# Autodesk Inventor assembly: ExtruderQuickReleaseRight
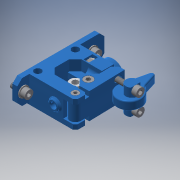
[picture p0: Inventor's stored thumbnail of the model, 180x180]
Saved by Autodesk Inventor 2016 (Build 200138000, 138)
## iProperties
Created: 2015-05-07
Part Number: ExtruderQuickReleaseRight
Document SubType Name: Assembly
Designer: Jack
Author: Jack
## Documents named in this file (14)
- C:\Users\Jack\ownCloud\Projects\CrossBot\InventorModel\Extruder\ExtruderQuickRelease\ExtruderQuickReleaseRight.iam
- C:\Users\Jack\ownCloud\Projects\CrossBot\InventorModel\Extruder\ExtruderQuickRelease\ExtruderQuickReleaseBodyRight.ipt
- C:\Users\Jack\ownCloud\Projects\CrossBot\InventorModel\Extruder\ExtruderQuickRelease\ExtruderQuickReleaseIdlerRight.ipt
- C:\Users\Jack\ownCloud\Projects\CrossBot\InventorModel\Extruder\ExtruderQuickRelease\ExtruderQuickReleaseTensionCam.ipt
- C:\Users\Jack\ownCloud\Projects\CrossBot\InventorModel\Extruder\ExtruderQuickRelease\ExtruderQuickReleaseTensionDowel.ipt
- C:\Users\Jack\ownCloud\Projects\CrossBot\InventorModel\Electronics\Motors\StepperMotorNema17x60mm.ipt
- C:\Users\Jack\ownCloud\Projects\CrossBot\InventorModel\Hardware\Extruder\DriveGearMK8.ipt
- C:\Users\Jack\ownCloud\Projects\CrossBot\InventorModel\Hardware\Bearing\BearingRadialBall\BearingRadialBall624zz.ipt
- C:\Users\Jack\ownCloud\Projects\CrossBot\InventorModel\Hardware\Nuts\Nut4.ipt
- C:\Users\Jack\ownCloud\Projects\CrossBot\InventorModel\Hardware\BoltWashers\BoltWasher4\BoltWasher4x10.iam
- C:\Users\Jack\ownCloud\Projects\CrossBot\InventorModel\Hardware\Bolts\SHCS\SHCS3\SHCS3x10.ipt
- C:\Users\Jack\ownCloud\Projects\CrossBot\InventorModel\Hardware\Bolts\SHCS\SHCS3\SHCS3x20.ipt
- C:\Users\Jack\ownCloud\Projects\CrossBot\InventorModel\Hardware\Bolts\SHCS\SHCS4\SHCS4x14.ipt
- C:\Users\Jack\ownCloud\Projects\CrossBot\InventorModel\Hardware\Bolts\SHCS\SHCS4\SHCS4x40.ipt
## Components (18 placed, 13 different names)
1. ExtruderQuickReleaseBodyRight:1 — Mate:3, Mate:4, Mate:5, Mate:6, Mate:7, Mate:12, Mate:13, Mate:14, Mate:15, Mate:16, Mate:17, Mate:21, Mate:22, Angle:2, Angle:3, Mate:23, Mate:24, Mate:29, Mate:30, Mate:31, Mate:32
2. ExtruderQuickReleaseIdlerRight:1 — Mate:6, Mate:7, Mate:8, Mate:9, Mate:11, Mate:19, Angle:1, Tangent:1
3. ExtruderQuickReleaseTensionCam:1 — Mate:28, Flush:2, Tangent:1
4. ExtruderQuickReleaseTensionDowel:1 — Mate:26, Mate:27, Mate:28, Flush:2, Mate:33, Mate:34
5. StepperMotorNema17x60mm:1 — Mate:3, Mate:4, Mate:5
6. DriveGearMK8:1
7. BearingRadialBall624zz:1 — Mate:8, Mate:9, Mate:10
8. Nut4:1 — Mate:22, Angle:2, Mate:25
9. BoltWasher4x10:1 [sub-assembly] — Mate:29, Mate:32
10. BoltWasher4x10:2 [sub-assembly] — Mate:30, Mate:31
11. SHCS3x10:1 — Mate:13, Mate:17
12. SHCS3x10:2 — Mate:12, Mate:16
13. SHCS3x20:1 — Mate:14, Mate:15
14. SHCS4x14:1 — Mate:10, Mate:11, Mate:18
15. SHCS4x40:1 — Mate:24, Mate:25, Mate:26, Mate:33
16. SHCS4x40:2 — Mate:20, Mate:23, Mate:27, Mate:34
17. Nut4:2 — Mate:20, Mate:21, Angle:3
18. Nut4:3 — Mate:18, Mate:19, Angle:1
## Relationships (40: Mate 34, Angle 3, Flush 2, Tangent 1)
- [Mate]: StepperMotorNema17x60mm:1 ↔ DriveGearMK8:1
- [Mate] (1 mm): StepperMotorNema17x60mm:1 ↔ DriveGearMK8:1
- [Flush] (-2 mm): Nut4:1 ↔ SHCS4x40:1
- Mate:3: ExtruderQuickReleaseBodyRight:1 ↔ StepperMotorNema17x60mm:1
- Mate:4: ExtruderQuickReleaseBodyRight:1 ↔ StepperMotorNema17x60mm:1
- Mate:5: ExtruderQuickReleaseBodyRight:1 ↔ StepperMotorNema17x60mm:1
- Mate:6: ExtruderQuickReleaseBodyRight:1 ↔ ExtruderQuickReleaseIdlerRight:1
- Mate:7 (0.2 mm): ExtruderQuickReleaseBodyRight:1 ↔ ExtruderQuickReleaseIdlerRight:1
- Mate:8: ExtruderQuickReleaseIdlerRight:1 ↔ BearingRadialBall624zz:1
- Mate:9: ExtruderQuickReleaseIdlerRight:1 ↔ BearingRadialBall624zz:1
- Mate:10: BearingRadialBall624zz:1 ↔ SHCS4x14:1
- Mate:11: ExtruderQuickReleaseIdlerRight:1 ↔ SHCS4x14:1
- Mate:12: ExtruderQuickReleaseBodyRight:1 ↔ SHCS3x10:2
- Mate:13: ExtruderQuickReleaseBodyRight:1 ↔ SHCS3x10:1
- Mate:14: ExtruderQuickReleaseBodyRight:1 ↔ SHCS3x20:1
- Mate:15: ExtruderQuickReleaseBodyRight:1 ↔ SHCS3x20:1
- Mate:16: ExtruderQuickReleaseBodyRight:1 ↔ SHCS3x10:2
- Mate:17: ExtruderQuickReleaseBodyRight:1 ↔ SHCS3x10:1
- Mate:18: SHCS4x14:1 ↔ Nut4:3
- Mate:19: ExtruderQuickReleaseIdlerRight:1 ↔ Nut4:3
- Angle:1 (0 deg): ExtruderQuickReleaseIdlerRight:1 ↔ Nut4:3
- Mate:20: SHCS4x40:2 ↔ Nut4:2
- Mate:21: ExtruderQuickReleaseBodyRight:1 ↔ Nut4:2
- Mate:22: ExtruderQuickReleaseBodyRight:1 ↔ Nut4:1
- Angle:2 (0 deg): ExtruderQuickReleaseBodyRight:1 ↔ Nut4:1
- Angle:3 (0 deg): ExtruderQuickReleaseBodyRight:1 ↔ Nut4:2
- Mate:23: ExtruderQuickReleaseBodyRight:1 ↔ SHCS4x40:2
- Mate:24: ExtruderQuickReleaseBodyRight:1 ↔ SHCS4x40:1
- Mate:25: Nut4:1 ↔ SHCS4x40:1
- Mate:26: ExtruderQuickReleaseTensionDowel:1 ↔ SHCS4x40:1
- Mate:27: ExtruderQuickReleaseTensionDowel:1 ↔ SHCS4x40:2
- Mate:28: ExtruderQuickReleaseTensionCam:1 ↔ ExtruderQuickReleaseTensionDowel:1
- Flush:2 (-7 mm): ExtruderQuickReleaseTensionCam:1 ↔ ExtruderQuickReleaseTensionDowel:1
- Mate:29: ExtruderQuickReleaseBodyRight:1 ↔ BoltWasher4x10:1
- Mate:30: ExtruderQuickReleaseBodyRight:1 ↔ BoltWasher4x10:2
- Mate:31: ExtruderQuickReleaseBodyRight:1 ↔ BoltWasher4x10:2
- Mate:32: ExtruderQuickReleaseBodyRight:1 ↔ BoltWasher4x10:1
- Mate:33: ExtruderQuickReleaseTensionDowel:1 ↔ SHCS4x40:1
- Mate:34: ExtruderQuickReleaseTensionDowel:1 ↔ SHCS4x40:2
- Tangent:1: ExtruderQuickReleaseIdlerRight:1 ↔ ExtruderQuickReleaseTensionCam:1
